# Autodesk Inventor assembly: Winch mount assenbly
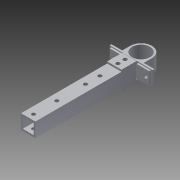
[picture p0: Inventor's stored thumbnail of the model, 180x180]
Saved by Autodesk Inventor 2013 (Build 170138000, 138)
## iProperties
Created: 2013-02-03
Part Number: Winch mount assenbly
Document SubType Name: Assembly
Designer: Arpan
Mass: 195.5 g
Surface Area: 482.628 cm^2
Volume: 72.1402 cm^3
Density: 2.71 g/cm^3
Author: Arpan
## Documents named in this file (4)
- C:\Users\Arpan\Documents\GitHub\frc2013CAD\Cimber actual\Winch mount assenbly.iam
- C:\Users\Arpan\Documents\GitHub\frc2013CAD\Cimber actual\winch mount.ipt
- C:\Users\Arpan\Documents\GitHub\frc2013CAD\Cimber actual\Winch mount frange.ipt
- C:\Users\Arpan\Documents\GitHub\frc2013CAD\Cimber actual\bearing mount.ipt
## Components (3 placed, 3 different names)
1. winch mount:1 — Mate:1, Mate:2, Flush:4
2. Winch mount frange:1 — Mate:1, Mate:2, Mate:3, Flush:2, Flush:3, Flush:4
3. bearing mount:1 — Mate:3, Flush:2, Flush:3
## Relationships (6: Mate 3, Flush 3)
- Mate:1: winch mount:1 ↔ Winch mount frange:1
- Mate:2: winch mount:1 ↔ Winch mount frange:1
- Mate:3: Winch mount frange:1 ↔ bearing mount:1
- Flush:2 (-3.175 mm): Winch mount frange:1 ↔ bearing mount:1
- Flush:3 (-1.5875 mm): Winch mount frange:1 ↔ bearing mount:1
- Flush:4: winch mount:1 ↔ Winch mount frange:1
